# Autodesk Inventor assembly: Gripper_Spindle
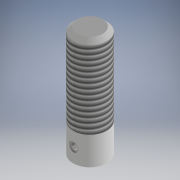
[picture p0: Inventor's stored thumbnail of the model, 180x180]
Saved by Autodesk Inventor 2021.3 (Build 253353000, 353)
## iProperties
Created: 2021-04-22
Part Number: Gripper_Spindle
Document SubType Name: Assembly
Designer: domin
Author: domin
## Documents named in this file (3)
- E:\Transfer\Sync\Hivemind\1-MCI-Unterlagen\Master\Semester 2\Projekt 1\Hausberger\Workfolder_Dommy\Gripper\Gripper_Spindle.iam
- E:\Transfer\Sync\Hivemind\1-MCI-Unterlagen\Master\Semester 2\Projekt 1\Hausberger\Workfolder_Dommy\Gripper\Spindle Iso M12 Setscrew.ipt
- C:\Users\domin\Documents\Inventor\Content Center Files\R2021\en-US\ISO 4026\ISO 4026 - M4 x 4 - ISO.ipt
## Components (2 placed, 2 different names)
1. Spindle Iso M12 Setscrew:1 — Mate:1, Mate:2, Mate:3, Mate:4, Flush:1
2. ISO 4026 M4 x 4:1 — Mate:4, Flush:1
## Relationships (5: Mate 4, Flush 1)
- Mate:1: Spindle Iso M12 Setscrew:1
- Mate:2: Spindle Iso M12 Setscrew:1
- Mate:3: Spindle Iso M12 Setscrew:1
- Mate:4: Spindle Iso M12 Setscrew:1 ↔ ISO 4026 M4 x 4:1
- Flush:1 (1.5 mm): Spindle Iso M12 Setscrew:1 ↔ ISO 4026 M4 x 4:1
